# Autodesk Inventor assembly: Backhoe
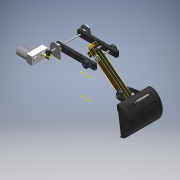
[picture p0: Inventor's stored thumbnail of the model, 180x180]
Saved by Autodesk Inventor 2019 (Build 230136000, 136)
## iProperties
Created: 2018-10-28
Part Number: Backhoe
Document SubType Name: Assembly
Designer: Alex Barnett
Author: Alex Barnett
## Documents named in this file (16)
- C:\Users\Alex Barnett\Documents\Machine Design\PR2\CAD\Backhoe.iam
- C:\Users\Alex Barnett\Documents\Machine Design\PR2\CAD\Boom Hinge.ipt
- C:\Users\Alex Barnett\Documents\Machine Design\PR2\CAD\Pin .5in. Dia. - Boom Hinge.ipt
- C:\Users\Alex Barnett\Documents\Machine Design\PR2\CAD\Ball Bearing .5in..ipt
- C:\Users\Alex Barnett\Documents\Machine Design\PR2\CAD\Steel 4130 1x2in. Tubing, t=.065in.,L=15in..ipt
- C:\Users\Alex Barnett\Documents\Machine Design\PR2\CAD\Flange-Mount Shaft Collar 0.5in..ipt
- C:\Users\Alex Barnett\Documents\Machine Design\PR2\CAD\Steel 4130 1x2in. Tubing, t=.065in.,L=22in..ipt
- C:\Users\Alex Barnett\Documents\Machine Design\PR2\CAD\Flange-Mount Sealed Ball Bearing .5in. Dia..ipt
- C:\Users\Alex Barnett\Documents\Machine Design\PR2\CAD\Boom to Stick .5in. Pin.ipt
- C:\Users\Alex Barnett\Documents\Machine Design\PR2\CAD\AmpFlow Motor & Gearbox.iam
- C:\Users\Alex Barnett\Documents\Machine Design\PR2\CAD\Worm Gear 12P 18T.ipt
- C:\Users\Alex Barnett\Documents\Machine Design\PR2\CAD\Steel 4130 1x2in. Tubing, t=.065in.,L=22in. Mirrored.ipt
- C:\Users\Alex Barnett\Documents\Machine Design\PR2\CAD\Stick to Scoop .5in. Pin.ipt
- C:\Users\Alex Barnett\Documents\Machine Design\PR2\CAD\Bucket.ipt
- C:\Users\Alex Barnett\Documents\Machine Design\PR2\CAD\Linear Actuator Top Pin .5in. Dia..ipt
- C:\Users\Alex Barnett\Documents\Machine Design\PR2\CAD\Linear Actuator Top Scoop Pin .5in. Dia..ipt
## Components (25 placed, 15 different names)
1. Boom Hinge:1 — Mate:1, Mate:2, Mate:3, Flush:2, Mate:6, Mate:7, Flush:3, Mate:14, Mate:26
2. Boom Hinge:2 — Mate:5, Flush:2, Mate:8, Flush:4, Flush:5, Mate:14, Mate:19, Mate:54, Flush:11
3. Pin .5in. Dia. - Boom Hinge:1 — Mate:5, Mate:6, Flush:5, Mate:15, Mate:21, Mate:22, Mate:54, Mate:67, Mate:68, Flush:16, Flush:23
4. Ball Bearing .5in.:1 — Mate:7, Flush:3
5. Ball Bearing .5in.:2 — Mate:8, Flush:4
6. Steel 4130 1x2in. Tubing, t=.065in.,L=15in.:1 — Flush:6, Mate:21, Mate:23, Mate:24, Mate:32, Mate:33, Mate:34, Flush:23
7. Flange-Mount Shaft Collar 0.5in.:2 — Mate:15, Mate:16, Mate:17, Mate:18, Mate:19
8. Steel 4130 1x2in. Tubing, t=.065in.,L=15in.:2 — Mate:16, Mate:17, Mate:18, Flush:6, Mate:29, Mate:30, Mate:31
9. Flange-Mount Shaft Collar 0.5in.:3 — Mate:22, Mate:23, Mate:24, Mate:26
10. Flange-Mount Sealed Ball Bearing .5in. Dia.:1 — Mate:29, Mate:30, Mate:31, Mate:35, Flush:8
11. Flange-Mount Sealed Ball Bearing .5in. Dia.:2 — Mate:32, Mate:33, Mate:34
12. Boom to Stick .5in. Pin:1 — Mate:35, Flush:8, Mate:72, Mate:73, Mate:74, Mate:80, Mate:81
13. AmpFlow Motor & Gearbox:1 [sub-assembly] — Mate:69, Mate:70, Mate:71
14. Worm Gear 12P 18T:1 — Mate:67, Mate:68, Flush:16, Mate:69, Mate:70, Mate:71
15. Steel 4130 1x2in. Tubing, t=.065in.,L=22in.:1 — Mate:72, Mate:73, Mate:75, Mate:76, Mate:77, Mate:78, Mate:79, Flush:17, Mate:84, Flush:19, Mate:95
16. Flange-Mount Shaft Collar 0.5in.:4 — Mate:74, Mate:75, Mate:76
17. Flange-Mount Sealed Ball Bearing .5in. Dia.:3 — Mate:77, Mate:78, Mate:79
18. Steel 4130 1x2in. Tubing, t=.065in.,L=22in. Mirrored:1 — Mate:80, Flush:17, Mate:82, Mate:83, Mate:84, Mate:85, Mate:86, Mate:87, Flush:18, Mate:91, Flush:21, Flush:22
19. Flange-Mount Shaft Collar 0.5in.:5 — Mate:81, Mate:82, Mate:83
20. Flange-Mount Sealed Ball Bearing .5in. Dia.:4 — Mate:85, Mate:86, Mate:87, Mate:88
21. Stick to Scoop .5in. Pin:1 — Mate:88, Flush:18, Mate:89
22. Bucket:1 — Mate:89, Flush:19, Mate:93, Mate:94
23. Linear Actuator Top Pin .5in. Dia.:1 — Mate:91, Flush:21
24. Linear Actuator Top Scoop Pin .5in. Dia.:1 — Mate:93, Mate:94
25. Linear Actuator Top Pin .5in. Dia.:2 — Mate:95, Flush:22
## Relationships (69: Mate 53, Flush 16)
- Mate:1: Boom Hinge:1
- Mate:2: Boom Hinge:1
- Mate:3: Boom Hinge:1
- Mate:5: Boom Hinge:2 ↔ Pin .5in. Dia. - Boom Hinge:1
- Flush:2: Boom Hinge:1 ↔ Boom Hinge:2
- Mate:6: Boom Hinge:1 ↔ Pin .5in. Dia. - Boom Hinge:1
- Mate:7: Boom Hinge:1 ↔ Ball Bearing .5in.:1
- Flush:3: Boom Hinge:1 ↔ Ball Bearing .5in.:1
- Mate:8: Boom Hinge:2 ↔ Ball Bearing .5in.:2
- Flush:4: Boom Hinge:2 ↔ Ball Bearing .5in.:2
- Flush:5: Boom Hinge:2 ↔ Pin .5in. Dia. - Boom Hinge:1
- Mate:14 (-304.8 mm): Boom Hinge:1 ↔ Boom Hinge:2
- Mate:15: Pin .5in. Dia. - Boom Hinge:1 ↔ Flange-Mount Shaft Collar 0.5in.:2
- Mate:16: Flange-Mount Shaft Collar 0.5in.:2 ↔ Steel 4130 1x2in. Tubing, t=.065in.,L=15in.:2
- Mate:17: Flange-Mount Shaft Collar 0.5in.:2 ↔ Steel 4130 1x2in. Tubing, t=.065in.,L=15in.:2
- Mate:18: Flange-Mount Shaft Collar 0.5in.:2 ↔ Steel 4130 1x2in. Tubing, t=.065in.,L=15in.:2
- Flush:6: Steel 4130 1x2in. Tubing, t=.065in.,L=15in.:1 ↔ Steel 4130 1x2in. Tubing, t=.065in.,L=15in.:2
- Mate:19 (6.35 mm): Boom Hinge:2 ↔ Flange-Mount Shaft Collar 0.5in.:2
- Mate:21: Pin .5in. Dia. - Boom Hinge:1 ↔ Steel 4130 1x2in. Tubing, t=.065in.,L=15in.:1
- Mate:22: Pin .5in. Dia. - Boom Hinge:1 ↔ Flange-Mount Shaft Collar 0.5in.:3
- Mate:23: Steel 4130 1x2in. Tubing, t=.065in.,L=15in.:1 ↔ Flange-Mount Shaft Collar 0.5in.:3
- Mate:24: Steel 4130 1x2in. Tubing, t=.065in.,L=15in.:1 ↔ Flange-Mount Shaft Collar 0.5in.:3
- Mate:26 (6.35 mm): Boom Hinge:1 ↔ Flange-Mount Shaft Collar 0.5in.:3
- Mate:29: Steel 4130 1x2in. Tubing, t=.065in.,L=15in.:2 ↔ Flange-Mount Sealed Ball Bearing .5in. Dia.:1
- Mate:30: Steel 4130 1x2in. Tubing, t=.065in.,L=15in.:2 ↔ Flange-Mount Sealed Ball Bearing .5in. Dia.:1
- Mate:31: Steel 4130 1x2in. Tubing, t=.065in.,L=15in.:2 ↔ Flange-Mount Sealed Ball Bearing .5in. Dia.:1
- Mate:32: Steel 4130 1x2in. Tubing, t=.065in.,L=15in.:1 ↔ Flange-Mount Sealed Ball Bearing .5in. Dia.:2
- Mate:33: Steel 4130 1x2in. Tubing, t=.065in.,L=15in.:1 ↔ Flange-Mount Sealed Ball Bearing .5in. Dia.:2
- Mate:34: Steel 4130 1x2in. Tubing, t=.065in.,L=15in.:1 ↔ Flange-Mount Sealed Ball Bearing .5in. Dia.:2
- Mate:35: Flange-Mount Sealed Ball Bearing .5in. Dia.:1 ↔ Boom to Stick .5in. Pin:1
- Flush:8: Flange-Mount Sealed Ball Bearing .5in. Dia.:1 ↔ Boom to Stick .5in. Pin:1
- Mate:54: Boom Hinge:2 ↔ Pin .5in. Dia. - Boom Hinge:1
- Flush:11: Boom Hinge:2
- Flush:12 (300 mm)
- Flush:13 (500 mm)
- Mate:67: Pin .5in. Dia. - Boom Hinge:1 ↔ Worm Gear 12P 18T:1
- Mate:68: Pin .5in. Dia. - Boom Hinge:1 ↔ Worm Gear 12P 18T:1
- Flush:16: Pin .5in. Dia. - Boom Hinge:1 ↔ Worm Gear 12P 18T:1
- Mate:69: AmpFlow Motor & Gearbox:1 ↔ Worm Gear 12P 18T:1
- Mate:70: AmpFlow Motor & Gearbox:1 ↔ Worm Gear 12P 18T:1
- Mate:71: AmpFlow Motor & Gearbox:1 ↔ Worm Gear 12P 18T:1
- Mate:72: Boom to Stick .5in. Pin:1 ↔ Steel 4130 1x2in. Tubing, t=.065in.,L=22in.:1
- Mate:73: Boom to Stick .5in. Pin:1 ↔ Steel 4130 1x2in. Tubing, t=.065in.,L=22in.:1
- Mate:74: Boom to Stick .5in. Pin:1 ↔ Flange-Mount Shaft Collar 0.5in.:4
- Mate:75: Steel 4130 1x2in. Tubing, t=.065in.,L=22in.:1 ↔ Flange-Mount Shaft Collar 0.5in.:4
- Mate:76: Steel 4130 1x2in. Tubing, t=.065in.,L=22in.:1 ↔ Flange-Mount Shaft Collar 0.5in.:4
- Mate:77: Steel 4130 1x2in. Tubing, t=.065in.,L=22in.:1 ↔ Flange-Mount Sealed Ball Bearing .5in. Dia.:3
- Mate:78: Steel 4130 1x2in. Tubing, t=.065in.,L=22in.:1 ↔ Flange-Mount Sealed Ball Bearing .5in. Dia.:3
- Mate:79: Steel 4130 1x2in. Tubing, t=.065in.,L=22in.:1 ↔ Flange-Mount Sealed Ball Bearing .5in. Dia.:3
- Mate:80: Boom to Stick .5in. Pin:1 ↔ Steel 4130 1x2in. Tubing, t=.065in.,L=22in. Mirrored:1
- Flush:17: Steel 4130 1x2in. Tubing, t=.065in.,L=22in.:1 ↔ Steel 4130 1x2in. Tubing, t=.065in.,L=22in. Mirrored:1
- Mate:81: Boom to Stick .5in. Pin:1 ↔ Flange-Mount Shaft Collar 0.5in.:5
- Mate:82: Steel 4130 1x2in. Tubing, t=.065in.,L=22in. Mirrored:1 ↔ Flange-Mount Shaft Collar 0.5in.:5
- Mate:83: Steel 4130 1x2in. Tubing, t=.065in.,L=22in. Mirrored:1 ↔ Flange-Mount Shaft Collar 0.5in.:5
- Mate:84: Steel 4130 1x2in. Tubing, t=.065in.,L=22in.:1 ↔ Steel 4130 1x2in. Tubing, t=.065in.,L=22in. Mirrored:1
- Mate:85: Steel 4130 1x2in. Tubing, t=.065in.,L=22in. Mirrored:1 ↔ Flange-Mount Sealed Ball Bearing .5in. Dia.:4
- Mate:86: Steel 4130 1x2in. Tubing, t=.065in.,L=22in. Mirrored:1 ↔ Flange-Mount Sealed Ball Bearing .5in. Dia.:4
- Mate:87: Steel 4130 1x2in. Tubing, t=.065in.,L=22in. Mirrored:1 ↔ Flange-Mount Sealed Ball Bearing .5in. Dia.:4
- Mate:88: Flange-Mount Sealed Ball Bearing .5in. Dia.:4 ↔ Stick to Scoop .5in. Pin:1
- Flush:18: Steel 4130 1x2in. Tubing, t=.065in.,L=22in. Mirrored:1 ↔ Stick to Scoop .5in. Pin:1
- Mate:89: Stick to Scoop .5in. Pin:1 ↔ Bucket:1
- Flush:19: Steel 4130 1x2in. Tubing, t=.065in.,L=22in.:1 ↔ Bucket:1
- Mate:91: Steel 4130 1x2in. Tubing, t=.065in.,L=22in. Mirrored:1 ↔ Linear Actuator Top Pin .5in. Dia.:1
- Flush:21: Steel 4130 1x2in. Tubing, t=.065in.,L=22in. Mirrored:1 ↔ Linear Actuator Top Pin .5in. Dia.:1
- Mate:93: Bucket:1 ↔ Linear Actuator Top Scoop Pin .5in. Dia.:1
- Mate:94: Bucket:1 ↔ Linear Actuator Top Scoop Pin .5in. Dia.:1
- Mate:95: Steel 4130 1x2in. Tubing, t=.065in.,L=22in.:1 ↔ Linear Actuator Top Pin .5in. Dia.:2
- Flush:22: Steel 4130 1x2in. Tubing, t=.065in.,L=22in. Mirrored:1 ↔ Linear Actuator Top Pin .5in. Dia.:2
- Flush:23: Pin .5in. Dia. - Boom Hinge:1 ↔ Steel 4130 1x2in. Tubing, t=.065in.,L=15in.:1
